# Autodesk Inventor assembly: MotorEsOrsoHajtas
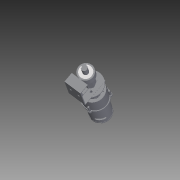
[picture p0: Inventor's stored thumbnail of the model, 180x180]
Saved by Autodesk Inventor 2015 (Build 190159000, 159)
## iProperties
Created: 2014-10-20
Part Number: MotorEsOrsoHajtas
Document SubType Name: Assembly
Designer: laca
Author: laca
## Documents named in this file (6)
- C:\Users\laca\Desktop\iRoobo2014Ver3\MotorKerekHajtas.iam
- C:\Users\laca\Desktop\iRoobo2014Ver3\MotorTartoElso.ipt
- C:\Users\laca\Desktop\iRoobo2014Ver3\Csapagy6900.ipt
- C:\Users\laca\Desktop\iRoobo2014Ver3\Biztositek15mm.ipt
- C:\Users\laca\Desktop\iRoobo2014Ver3\Motor.iam
- C:\Users\laca\Desktop\iRoobo2014Ver3\AnyaKicsiOldalso.ipt
## Components (5 placed, 5 different names)
1. MotorTartoElso:1 — Rigid:1, Insert:5, Insert:6
2. Csapagy6900:2 — Rigid:1, Cylindrical:6
3. Biztositek15mm:2 — Cylindrical:4, Cylindrical:5, Flush:1
4. Motor:1 [sub-assembly] — Insert:5, Cylindrical:4, Insert:6
5. AnyaKicsiOldalso:1 — Cylindrical:5, Cylindrical:6, Flush:1
## Relationships (7: CylindricalJoint 3, Insert 2, WeldJoint 1, Flush 1)
- Rigid:1 [WeldJoint]: MotorTartoElso:1 ↔ Csapagy6900:2
- Insert:5: MotorTartoElso:1 ↔ Motor:1
- Cylindrical:4: Biztositek15mm:2 ↔ Motor:1
- Insert:6: MotorTartoElso:1 ↔ Motor:1
- Cylindrical:5: Biztositek15mm:2 ↔ AnyaKicsiOldalso:1
- Cylindrical:6: Csapagy6900:2 ↔ AnyaKicsiOldalso:1
- Flush:1: Biztositek15mm:2 ↔ AnyaKicsiOldalso:1
